# Autodesk Inventor assembly: Micropippete mount assembly
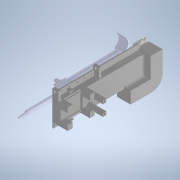
[picture p0: Inventor's stored thumbnail of the model, 180x180]
Saved by Autodesk Inventor 2022 (Build 260153000, 153)
## iProperties
Created: 2021-10-07
Part Number: Micropippete mount assembly
Document SubType Name: Assembly
Designer: efred
Sending System: Autodesk Translation Framework v10.10.0.1391
Preprocessor: ST-DEVELOPER v18.1
Title: /Users/sarthakdas/Downloads/Micropippete mount v12.step
## Documents named in this file (5)
- C:\Users\efred\OneDrive - Imperial College London\ROBOICP\Final Assembly\Micropippete mount assembly.iam
- C:\Users\efred\OneDrive - Imperial College London\ROBOICP\Old Files\roboICP-main\Sarthaks CAD Files\Part2.ipt
- C:\Users\efred\OneDrive - Imperial College London\ROBOICP\Final Assembly\Body Pippete Holder v2.ipt
- C:\Users\efred\OneDrive - Imperial College London\ROBOICP\Final Assembly\Micropipette.ipt
- C:\Users\efred\OneDrive - Imperial College London\ROBOICP\Final Assembly\big servo.ipt
## Components (5 placed, 4 different names)
1. Part2 — Angle:1, Mate:1, Mate:2, Mate:3, Mate:4, Mate:5, Mate:6, Mate:7, Flush:2, Mate:10, Mate:11, Mate:12
2. Micropipette:1 — Angle:1, Flush:1, Flush:2, Mate:10
3. big servo:1 — Mate:1, Mate:2, Mate:3
4. big servo:2 — Mate:4, Mate:5, Mate:6
5. Body Pippete Holder v2:1 — Mate:7, Flush:1, Mate:11, Mate:12
## Relationships (13: Mate 10, Flush 2, Angle 1)
- Angle:1 (0 deg): Part2 ↔ Micropipette:1
- Mate:1 (0.1 mm): Part2 ↔ big servo:1
- Mate:2 (0.1 mm): Part2 ↔ big servo:1
- Mate:3: Part2 ↔ big servo:1
- Mate:4: Part2 ↔ big servo:2
- Mate:5: Part2 ↔ big servo:2
- Mate:6: Part2 ↔ big servo:2
- Mate:7: Part2 ↔ Body Pippete Holder v2:1
- Flush:1: Micropipette:1 ↔ Body Pippete Holder v2:1
- Flush:2 (-18.5 mm): Part2 ↔ Micropipette:1
- Mate:10 (7 mm): Part2 ↔ Micropipette:1
- Mate:11: Part2 ↔ Body Pippete Holder v2:1
- Mate:12: Part2 ↔ Body Pippete Holder v2:1
